# Autodesk Inventor assembly: Tamale - V1p5
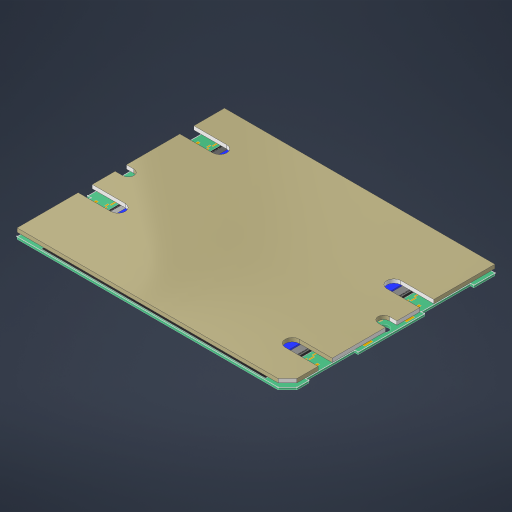
[picture p0: Inventor's stored thumbnail of the model, 512x512]
Saved by Autodesk Inventor 2024 (Build 280153000, 153)
## iProperties
Created: 2023-01-11
Part Number: Tamale - V1p5
Document SubType Name: Assembly
Designer: Caleb
Author: Caleb
## Documents named in this file (7)
- C:\Users\cfangmeier3\Desktop\nebraska-silicon-lab\Hardware\ETL\modules\tamale v1.5\Tamale - V1p5.iam
- C:\Users\cfangmeier3\Desktop\nebraska-silicon-lab\Hardware\ETL\modules\tamale v1.5\Baseplate v1.5.ipt
- C:\Users\cfangmeier3\Desktop\nebraska-silicon-lab\Hardware\ETL\modules\tamale v1.5\etl_module_pcb_mockup_v3p3p1.ipt
- C:\Users\cfangmeier3\Desktop\nebraska-silicon-lab\Hardware\ETL\modules\tamale v1.5\Sensor Placement Film.ipt
- C:\Users\cfangmeier3\Desktop\nebraska-silicon-lab\Hardware\ETL\modules\tamale v1.5\BBM.iam
- C:\Users\cfangmeier3\Desktop\nebraska-silicon-lab\Hardware\ETL\modules\tamale v1.5\Coverplate Film.ipt
- C:\Users\cfangmeier3\Desktop\nebraska-silicon-lab\Hardware\ETL\modules\tamale v1.5\Thermal Pad.ipt
## Components (9 placed, 6 different names)
1. Baseplate v1.5:1 — Mate:9, Flush:10, Flush:11, Mate:10, Flush:12, Flush:13
2. etl_module_pcb_mockup_v3p3p1:1 — Mate:1, Flush:1, Flush:2, Flush:10, Flush:11
3. Sensor Placement Film:1 — Mate:1, Flush:1, Flush:2, Mate:2, Mate:3, Mate:4, Mate:5, Flush:3, Flush:8
4. BBM:1 [sub-assembly] — Mate:2, Flush:4, Mate:6, Flush:6
5. BBM:2 [sub-assembly] — Mate:5, Flush:3, Flush:4, Mate:6, Mate:7, Flush:5, Flush:8, Mate:8
6. BBM:3 [sub-assembly] — Mate:4, Flush:6, Flush:7
7. BBM:4 [sub-assembly] — Mate:3, Mate:7, Flush:5, Flush:7, Flush:9
8. Coverplate Film:1 — Mate:8, Flush:9, Mate:9
9. Thermal Pad:1 — Mate:10, Flush:12, Flush:13
## Relationships (23: Flush 13, Mate 10)
- Mate:1: etl_module_pcb_mockup_v3p3p1:1 ↔ Sensor Placement Film:1
- Flush:1 (0.25 mm): etl_module_pcb_mockup_v3p3p1:1 ↔ Sensor Placement Film:1
- Flush:2 (4.95 mm): etl_module_pcb_mockup_v3p3p1:1 ↔ Sensor Placement Film:1
- Mate:2: Sensor Placement Film:1 ↔ BBM:1
- Mate:3: Sensor Placement Film:1 ↔ BBM:4
- Mate:4: Sensor Placement Film:1 ↔ BBM:3
- Mate:5: Sensor Placement Film:1 ↔ BBM:2
- Flush:3 (0.5 mm): Sensor Placement Film:1 ↔ BBM:2
- Flush:4: BBM:1 ↔ BBM:2
- Mate:6 (0.2 mm): BBM:1 ↔ BBM:2
- Mate:7 (0.2 mm): BBM:2 ↔ BBM:4
- Flush:5: BBM:2 ↔ BBM:4
- Flush:6: BBM:1 ↔ BBM:3
- Flush:7: BBM:3 ↔ BBM:4
- Flush:8 (0.5 mm): Sensor Placement Film:1 ↔ BBM:2
- Mate:8: BBM:2 ↔ Coverplate Film:1
- Flush:9 (0.5 mm): BBM:4 ↔ Coverplate Film:1
- Mate:9: Baseplate v1.5:1 ↔ Coverplate Film:1
- Flush:10: Baseplate v1.5:1 ↔ etl_module_pcb_mockup_v3p3p1:1
- Flush:11: Baseplate v1.5:1 ↔ etl_module_pcb_mockup_v3p3p1:1
- Mate:10: Baseplate v1.5:1 ↔ Thermal Pad:1
- Flush:12 (0.5 mm): Baseplate v1.5:1 ↔ Thermal Pad:1
- Flush:13 (0.5 mm): Baseplate v1.5:1 ↔ Thermal Pad:1
